# Autodesk Inventor assembly: Барабан сборка
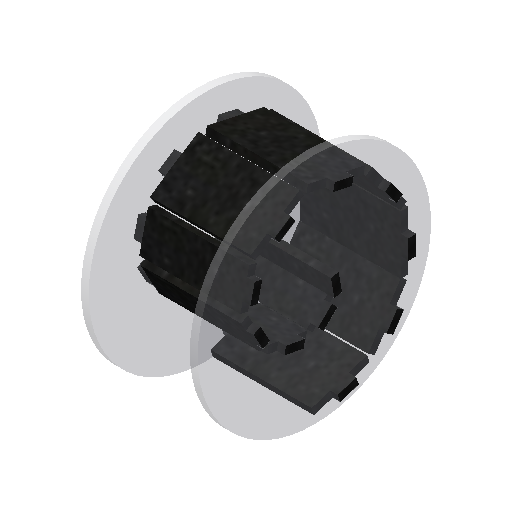
[picture p0: Inventor's stored thumbnail of the model, 512x512]
Saved by Autodesk Inventor 2022 (Build 260153000, 153)
## iProperties
Created: 2023-02-13
Part Number: Барабан сборка
Document SubType Name: Assembly
Designer: Глеб
Mass: 145.598 g
Surface Area: 856.789 cm^2
Volume: 145.598 cm^3
Density: 1 g/cm^3
Author: Глеб
## Documents named in this file (6)
- C:\Users\Глеб\Documents\Inventor\Файлы Inventor\Барабан сборка.iam
- C:\Users\Глеб\Documents\Inventor\Файлы Inventor\Стенка барабана.ipt
- C:\Users\Глеб\Documents\Inventor\Файлы Inventor\Кусочек барабана 30 мм.ipt
- C:\Users\Глеб\Documents\Inventor\Файлы Inventor\Кусочек барабана 20 мм.ipt
- C:\Users\Глеб\Documents\Inventor\Файлы Inventor\Кусочек барабана 15 мм.ipt
- C:\Users\Глеб\Documents\Inventor\Файлы Inventor\Кусочек барабана 10 мм.ipt
## Components (13 placed, 5 different names)
1. Стенка барабана:1 — Совмещение:7, Совмещение:8, Совмещение:9, Совмещение:10, Совмещение:11, Совмещение:12, Совмещение:13, Совмещение:14, Совмещение:15, Совмещение:16, Совмещение:17, Совмещение:18, Совмещение:19, Совмещение:20, Совмещение:21, Совмещение:22, Совмещение:23, Совмещение:24, Совмещение:30, Совмещение:31, Совмещение:32, Совмещение:33, Совмещение:34, Совмещение:35, Совмещение:36, Совмещение:37, Совмещение:38, Совмещение:46, Совмещение:47, Совмещение:49, Совмещение:50
2. Кусочек барабана 30 мм:1 — Совмещение:7, Совмещение:8, Совмещение:9, Совмещение:42, Совмещение:43, Совмещение:44
3. Кусочек барабана 30 мм:2 — Совмещение:10, Совмещение:11, Совмещение:12
4. Кусочек барабана 30 мм:3 — Совмещение:13, Совмещение:14, Совмещение:15
5. Кусочек барабана 30 мм:5 — Совмещение:16, Совмещение:17, Совмещение:18
6. Кусочек барабана 15 мм:1 — Совмещение:33, Совмещение:34, Совмещение:35
7. Кусочек барабана 30 мм:6 — Совмещение:19, Совмещение:20, Совмещение:21
8. Кусочек барабана 30 мм:7 — Совмещение:22, Совмещение:23, Совмещение:24
9. Кусочек барабана 20 мм:5 — Совмещение:30, Совмещение:31, Совмещение:32
10. Кусочек барабана 10 мм:1 — Совмещение:36, Совмещение:37, Совмещение:38
11. Стенка барабана:2 — Совмещение:42, Совмещение:43, Совмещение:44, Совмещение:45, Совмещение:48
12. Кусочек барабана 20 мм:6 — Совмещение:45, Совмещение:46, Совмещение:47
13. Кусочек барабана 20 мм:7 — Совмещение:48, Совмещение:49, Совмещение:50
## Relationships (36: Mate 36)
- Совмещение:7 [Mate]: Стенка барабана:1 ↔ Кусочек барабана 30 мм:1
- Совмещение:8 [Mate]: Стенка барабана:1 ↔ Кусочек барабана 30 мм:1
- Совмещение:9 [Mate]: Стенка барабана:1 ↔ Кусочек барабана 30 мм:1
- Совмещение:10 [Mate]: Стенка барабана:1 ↔ Кусочек барабана 30 мм:2
- Совмещение:11 [Mate]: Стенка барабана:1 ↔ Кусочек барабана 30 мм:2
- Совмещение:12 [Mate]: Стенка барабана:1 ↔ Кусочек барабана 30 мм:2
- Совмещение:13 [Mate]: Стенка барабана:1 ↔ Кусочек барабана 30 мм:3
- Совмещение:14 [Mate]: Стенка барабана:1 ↔ Кусочек барабана 30 мм:3
- Совмещение:15 [Mate]: Стенка барабана:1 ↔ Кусочек барабана 30 мм:3
- Совмещение:16 [Mate]: Стенка барабана:1 ↔ Кусочек барабана 30 мм:5
- Совмещение:17 [Mate]: Стенка барабана:1 ↔ Кусочек барабана 30 мм:5
- Совмещение:18 [Mate]: Стенка барабана:1 ↔ Кусочек барабана 30 мм:5
- Совмещение:19 [Mate]: Стенка барабана:1 ↔ Кусочек барабана 30 мм:6
- Совмещение:20 [Mate]: Стенка барабана:1 ↔ Кусочек барабана 30 мм:6
- Совмещение:21 [Mate]: Стенка барабана:1 ↔ Кусочек барабана 30 мм:6
- Совмещение:22 [Mate]: Стенка барабана:1 ↔ Кусочек барабана 30 мм:7
- Совмещение:23 [Mate]: Стенка барабана:1 ↔ Кусочек барабана 30 мм:7
- Совмещение:24 [Mate]: Стенка барабана:1 ↔ Кусочек барабана 30 мм:7
- Совмещение:30 [Mate]: Стенка барабана:1 ↔ Кусочек барабана 20 мм:5
- Совмещение:31 [Mate]: Стенка барабана:1 ↔ Кусочек барабана 20 мм:5
- Совмещение:32 [Mate]: Стенка барабана:1 ↔ Кусочек барабана 20 мм:5
- Совмещение:33 [Mate]: Стенка барабана:1 ↔ Кусочек барабана 15 мм:1
- Совмещение:34 [Mate]: Стенка барабана:1 ↔ Кусочек барабана 15 мм:1
- Совмещение:35 [Mate]: Стенка барабана:1 ↔ Кусочек барабана 15 мм:1
- Совмещение:36 [Mate]: Стенка барабана:1 ↔ Кусочек барабана 10 мм:1
- Совмещение:37 [Mate]: Стенка барабана:1 ↔ Кусочек барабана 10 мм:1
- Совмещение:38 [Mate]: Стенка барабана:1 ↔ Кусочек барабана 10 мм:1
- Совмещение:42 [Mate]: Кусочек барабана 30 мм:1 ↔ Стенка барабана:2
- Совмещение:43 [Mate]: Кусочек барабана 30 мм:1 ↔ Стенка барабана:2
- Совмещение:44 [Mate]: Кусочек барабана 30 мм:1 ↔ Стенка барабана:2
- Совмещение:45 [Mate]: Стенка барабана:2 ↔ Кусочек барабана 20 мм:6
- Совмещение:46 [Mate]: Стенка барабана:1 ↔ Кусочек барабана 20 мм:6
- Совмещение:47 [Mate]: Стенка барабана:1 ↔ Кусочек барабана 20 мм:6
- Совмещение:48 [Mate]: Стенка барабана:2 ↔ Кусочек барабана 20 мм:7
- Совмещение:49 [Mate]: Стенка барабана:1 ↔ Кусочек барабана 20 мм:7
- Совмещение:50 [Mate]: Стенка барабана:1 ↔ Кусочек барабана 20 мм:7
